# Autodesk Inventor assembly: Pierna
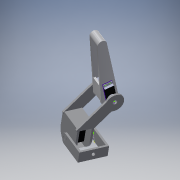
[picture p0: Inventor's stored thumbnail of the model, 180x180]
Saved by Autodesk Inventor 2018 (Build 220112000, 112)
## iProperties
Created: 2020-03-06
Part Number: Pierna
Document SubType Name: Assembly
Designer: GonzaloDiaz
Mass: 274.919 g
Surface Area: 1041.59 cm^2
Volume: 259.408 cm^3
Density: 1.05979 g/cm^3
Author: GonzaloDiaz
## Documents named in this file (7)
- E:\Universidad\Codigo\Enigma\Diseños\Pierna.iam
- E:\Universidad\Codigo\Enigma\Diseños\SERVOMG996R.ipt
- E:\Universidad\Codigo\Enigma\Diseños\Tibia.ipt
- E:\Universidad\Codigo\Enigma\Diseños\leva servo motore.ipt
- leva.ipt
- E:\Universidad\Codigo\Enigma\Diseños\Femur.ipt
- E:\Universidad\Codigo\Enigma\Diseños\Hombro.ipt
## Components (7 placed, 5 different names)
1. SERVOMG996R:1 — Insert:1, Mate:1, Mate:2, Mate:3
2. Tibia:1 — Mate:1, Mate:2, Mate:3, Insert:2, Rotational:1
3. leva:1 — Insert:1, Mate:7
4. Femur:1 — Insert:2, Mate:4, Mate:5, Mate:6, Mate:7, Insert:4, Rotational:1, Rotational:2
5. SERVOMG996R:2 — Mate:4, Mate:5, Mate:6, Insert:3
6. leva:2 — Insert:3, Flush:1
7. Hombro:1 — Insert:4, Rotational:2
## Relationships (14: Mate 7, Insert 4, RevoluteJoint 2, Flush 1)
- Insert:1: SERVOMG996R:1 ↔ leva:1
- Mate:1: SERVOMG996R:1 ↔ Tibia:1
- Mate:2: SERVOMG996R:1 ↔ Tibia:1
- Mate:3: SERVOMG996R:1 ↔ Tibia:1
- Insert:2: Tibia:1 ↔ Femur:1
- Mate:4: Femur:1 ↔ SERVOMG996R:2
- Mate:5: Femur:1 ↔ SERVOMG996R:2
- Mate:6: Femur:1 ↔ SERVOMG996R:2
- Insert:3: SERVOMG996R:2 ↔ leva:2
- Mate:7: leva:1 ↔ Femur:1
- Insert:4: Femur:1 ↔ Hombro:1
- Flush:1: leva:2
- Rotational:1 [RevoluteJoint]: Tibia:1 ↔ Femur:1
- Rotational:2 [RevoluteJoint]: Femur:1 ↔ Hombro:1
